# Autodesk Inventor assembly: Сборка1
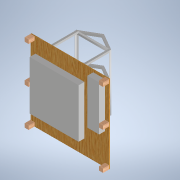
[picture p0: Inventor's stored thumbnail of the model, 180x180]
Saved by Autodesk Inventor 2022.4 (Build 264492010, 492A)
## iProperties
Created: 2023-02-19
Part Number: Сборка1
Document SubType Name: Assembly
Designer: artyo
Author: artyo
## Documents named in this file (13)
- C:\Users\artyo\OneDrive\Рабочий стол\ПРЕДПРОФ\Sborka1.iam
- C:\Users\artyo\OneDrive\Рабочий стол\ПРЕДПРОФ\columnnorm.ipt
- C:\Users\artyo\OneDrive\Рабочий стол\ПРЕДПРОФ\ОСНОВАФАНЕРА.ipt
- C:\Users\artyo\OneDrive\Рабочий стол\ПРЕДПРОФ\подпорка(МОЖНОМЕНЯТЬ).ipt
- C:\Users\artyo\OneDrive\Рабочий стол\ПРЕДПРОФ\Detal3.ipt
- C:\Users\artyo\OneDrive\Рабочий стол\ПРЕДПРОФ\Деталь2.ipt
- C:\Users\artyo\OneDrive\Рабочий стол\ПРЕДПРОФ\уголок 350.ipt
- C:\Users\artyo\OneDrive\Рабочий стол\ПРЕДПРОФ\уголок 580.ipt
- C:\Users\artyo\OneDrive\Рабочий стол\ПРЕДПРОФ\ЗЕМЛЯЕМКОСТЬ.ipt
- C:\Users\artyo\OneDrive\Рабочий стол\ПРЕДПРОФ\коробка ардуинкародина.ipt
- C:\Users\artyo\OneDrive\Рабочий стол\ПРЕДПРОФ\опора кинематик стенд.ipt
- C:\Users\artyo\OneDrive\Рабочий стол\ПРЕДПРОФ\Деталь8.ipt
- C:\Users\artyo\OneDrive\Рабочий стол\ПРЕДПРОФ\вал.ipt
## Components (32 placed, 12 different names)
1. ОСНОВАФАНЕРА:1 — Заподлицо:1, Совмещение:1, Заподлицо:2, Совмещение:4, Совмещение:5, Заподлицо:12, Заподлицо:13, Совмещение:6, Заподлицо:14, Совмещение:17, Заподлицо:19, Заподлицо:20, Совмещение:18, Совмещение:19, Заподлицо:21, Совмещение:20, Совмещение:22
2. Деталь2:1 — Совмещение:4, Совмещение:5, Заподлицо:12
3. уголок 580:1 — Заподлицо:16, Совмещение:9, Совмещение:10
4. уголок 580:2 — Заподлицо:17, Совмещение:11, Совмещение:12, Совмещение:13, Совмещение:14
5. ЗЕМЛЯЕМКОСТЬ:1 — Совмещение:15, Совмещение:16, Совмещение:17
6. коробка ардуинкародина:2 — Заподлицо:19, Заподлицо:20, Совмещение:18
7. опора кинематик стенд:1 — Совмещение:19, Заподлицо:21, Совмещение:20, Совмещение:21, Совмещение:23, Совмещение:24, Заподлицо:22, Совмещение:25
8. опора кинематик стенд:2 — Совмещение:21, Совмещение:22, Совмещение:23, Совмещение:26, Совмещение:27, Заподлицо:23, Совмещение:28, Заподлицо:26, Совмещение:30
9. Деталь8:1 — Совмещение:26, Совмещение:27, Заподлицо:23, Заподлицо:24, Заподлицо:25
10. Деталь8:2 — Совмещение:24, Заподлицо:22, Совмещение:25, Заподлицо:24, Заподлицо:25
11. вал:1 — Совмещение:28, Заподлицо:26, Совмещение:30
12. columnnorm:1 — Заподлицо:1, Совмещение:1, Заподлицо:2, Заподлицо:3
13. columnnorm:2 — Заподлицо:8, Совмещение:15
14. columnnorm:3 — Совмещение:10
15. columnnorm:4 — Совмещение:16
16. columnnorm:5 — Заподлицо:16
17. columnnorm:6 — Совмещение:7, Заподлицо:15, Совмещение:8, Заподлицо:17, Совмещение:12
18. Detal3:2 — Совмещение:2, Заподлицо:9
19. Detal3:1 — Совмещение:2, Заподлицо:9
20. Detal3:3
21. Detal3:4
22. Detal3:5
23. Detal3:6 — Совмещение:13, Совмещение:14, Заподлицо:18
24. подпорка(МОЖНОМЕНЯТЬ):1 — Заподлицо:13, Совмещение:6, Заподлицо:14
25. подпорка(МОЖНОМЕНЯТЬ):2
26. подпорка(МОЖНОМЕНЯТЬ):3
27. подпорка(МОЖНОМЕНЯТЬ):4
28. подпорка(МОЖНОМЕНЯТЬ):5
29. подпорка(МОЖНОМЕНЯТЬ):6
30. уголок 350:1 — Совмещение:7, Заподлицо:15, Совмещение:8, Совмещение:9, Совмещение:11, Заподлицо:18
31. уголок 350:2
32. уголок 350:3
## Component patterns: (6 elements, first: columnnorm:1), (3 elements, first: Detal3:2 + Detal3:1), (6 elements, first: подпорка(МОЖНОМЕНЯТЬ):1), (3 elements, first: уголок 350:1)
## Relationships (48: Mate 28, Flush 20)
- Заподлицо:1 [Flush] (100 mm): ОСНОВАФАНЕРА:1 ↔ columnnorm:1
- Совмещение:1 [Mate]: ОСНОВАФАНЕРА:1 ↔ columnnorm:1
- Заподлицо:2 [Flush] (100 mm): ОСНОВАФАНЕРА:1 ↔ columnnorm:1
- Заподлицо:3 [Flush] (-10 mm): columnnorm:1
- Заподлицо:8 [Flush] (-10 mm): columnnorm:2
- Совмещение:2 [Mate]: Detal3:2 ↔ Detal3:1
- Заподлицо:9 [Flush]: Detal3:2 ↔ Detal3:1
- Совмещение:4 [Mate]: ОСНОВАФАНЕРА:1 ↔ Деталь2:1
- Совмещение:5 [Mate] (-550 mm): ОСНОВАФАНЕРА:1 ↔ Деталь2:1
- Заподлицо:12 [Flush] (150 mm): ОСНОВАФАНЕРА:1 ↔ Деталь2:1
- Заподлицо:13 [Flush]: ОСНОВАФАНЕРА:1 ↔ подпорка(МОЖНОМЕНЯТЬ):1
- Совмещение:6 [Mate]: ОСНОВАФАНЕРА:1 ↔ подпорка(МОЖНОМЕНЯТЬ):1
- Заподлицо:14 [Flush]: ОСНОВАФАНЕРА:1 ↔ подпорка(МОЖНОМЕНЯТЬ):1
- Совмещение:7 [Mate]: columnnorm:6 ↔ уголок 350:1
- Заподлицо:15 [Flush]: columnnorm:6 ↔ уголок 350:1
- Совмещение:8 [Mate]: columnnorm:6 ↔ уголок 350:1
- Заподлицо:16 [Flush]: уголок 580:1 ↔ columnnorm:5
- Совмещение:9 [Mate]: уголок 580:1 ↔ уголок 350:1
- Совмещение:10 [Mate]: уголок 580:1 ↔ columnnorm:3
- Заподлицо:17 [Flush]: уголок 580:2 ↔ columnnorm:6
- Совмещение:11 [Mate]: уголок 580:2 ↔ уголок 350:1
- Совмещение:12 [Mate]: уголок 580:2 ↔ columnnorm:6
- Совмещение:13 [Mate]: уголок 580:2 ↔ Detal3:6
- Совмещение:14 [Mate]: уголок 580:2 ↔ Detal3:6
- Заподлицо:18 [Flush]: Detal3:6 ↔ уголок 350:1
- Совмещение:15 [Mate]: ЗЕМЛЯЕМКОСТЬ:1 ↔ columnnorm:2
- Совмещение:16 [Mate]: ЗЕМЛЯЕМКОСТЬ:1 ↔ columnnorm:4
- Совмещение:17 [Mate]: ОСНОВАФАНЕРА:1 ↔ ЗЕМЛЯЕМКОСТЬ:1
- Заподлицо:19 [Flush] (40 mm): ОСНОВАФАНЕРА:1 ↔ коробка ардуинкародина:2
- Заподлицо:20 [Flush] (20 mm): ОСНОВАФАНЕРА:1 ↔ коробка ардуинкародина:2
- Совмещение:18 [Mate]: ОСНОВАФАНЕРА:1 ↔ коробка ардуинкародина:2
- Совмещение:19 [Mate]: ОСНОВАФАНЕРА:1 ↔ опора кинематик стенд:1
- Заподлицо:21 [Flush] (50 mm): ОСНОВАФАНЕРА:1 ↔ опора кинематик стенд:1
- Совмещение:20 [Mate] (100.371 mm): ОСНОВАФАНЕРА:1 ↔ опора кинематик стенд:1
- Совмещение:21 [Mate] (100 mm): опора кинематик стенд:1 ↔ опора кинематик стенд:2
- Совмещение:22 [Mate]: ОСНОВАФАНЕРА:1 ↔ опора кинематик стенд:2
- Совмещение:23 [Mate] (4.145 mm): опора кинематик стенд:1 ↔ опора кинематик стенд:2
- Совмещение:24 [Mate]: опора кинематик стенд:1 ↔ Деталь8:2
- Заподлицо:22 [Flush]: опора кинематик стенд:1 ↔ Деталь8:2
- Совмещение:25 [Mate]: опора кинематик стенд:1 ↔ Деталь8:2
- Совмещение:26 [Mate]: опора кинематик стенд:2 ↔ Деталь8:1
- Совмещение:27 [Mate]: опора кинематик стенд:2 ↔ Деталь8:1
- Заподлицо:23 [Flush]: опора кинематик стенд:2 ↔ Деталь8:1
- Заподлицо:24 [Flush] (4.145 mm): Деталь8:1 ↔ Деталь8:2
- Заподлицо:25 [Flush]: Деталь8:1 ↔ Деталь8:2
- Совмещение:28 [Mate]: опора кинематик стенд:2 ↔ вал:1
- Заподлицо:26 [Flush]: опора кинематик стенд:2 ↔ вал:1
- Совмещение:30 [Mate]: опора кинематик стенд:2 ↔ вал:1
